# Autodesk Inventor assembly: Assembly6
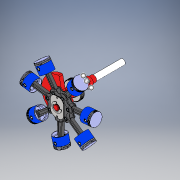
[picture p0: Inventor's stored thumbnail of the model, 180x180]
Saved by Autodesk Inventor 2018 (Build 220112000, 112)
## iProperties
Created: 2023-04-24
Part Number: Assembly6
Document SubType Name: Assembly
Designer: Habib Mohamed
Author: Habib Mohamed
## Documents named in this file (12)
- D:\Inventor\My projects\Rotary Engine\Assembly\Assembly6.iam
- D:\Inventor\My projects\Rotary Engine\Assembly\Assembly4 (Piston Sub Assembly).iam
- D:\Inventor\My projects\Rotary Engine\Component 2 (Connecting Rod Hub).ipt
- D:\Inventor\My projects\Rotary Engine\Component 31(Rod Axle).ipt
- D:\Inventor\My projects\Rotary Engine\Assembly\Assembly4 (Piston Sub Assembly Shrunk).iam
- D:\Inventor\My projects\Rotary Engine\Shaft.ipt
- D:\Inventor\My projects\Rotary Engine\Component 16 (Sun Wheel).ipt
- D:\Inventor\My projects\Rotary Engine\Component 17 (Feather Key).ipt
- D:\Inventor\My projects\Rotary Engine\Component 7 (Cover Plate).ipt
- C:\Users\Habib Mohamed\Documents\Inventor\Content Center Files\R2018\en-US\DIN 617 SKF(2)\DIN 617 SKF - SKF NA 4900 RS.ipt
- C:\Users\Habib Mohamed\Documents\Inventor\Content Center Files\R2018\en-US\DIN 6799\DIN 6799 - 9 10.ipt
- C:\Users\Habib Mohamed\Documents\Inventor\Content Center Files\R2018\en-US\DIN 6799\DIN 6799 - 10 11.ipt
## Components (21 placed, 11 different names)
1. Assembly4 (Piston Sub Assembly):1 [sub-assembly] — Mate:5, Mate:12
2. Component 2 (Connecting Rod Hub):1 — Mate:1, Mate:2, Mate:3, Mate:4, Mate:5, Mate:6, Mate:7, Mate:8, Mate:9, Mate:10, Mate:11, Mate:12, Mate:13, Mate:14, Mate:15, Mate:16, Mate:17, Mate:18, Mate:19, Mate:20, Flush:1, Flush:2, Flush:3, Flush:4, Flush:5, Mate:21, Mate:22, Mate:29, Mate:30, Flush:6, Mate:33, Mate:34
3. Component 31(Rod Axle):1 — Mate:18, Flush:1
4. Assembly4 (Piston Sub Assembly):2 [sub-assembly] — Mate:6, Mate:10
5. Assembly4 (Piston Sub Assembly):3 [sub-assembly] — Mate:7, Mate:11
6. Assembly4 (Piston Sub Assembly):4 [sub-assembly] — Mate:8, Mate:9
7. Assembly4 (Piston Sub Assembly):5 [sub-assembly] — Mate:4, Mate:13
8. Assembly4 (Piston Sub Assembly):6 [sub-assembly] — Mate:3, Mate:14
9. Assembly4 (Piston Sub Assembly Shrunk):1 [sub-assembly] — Mate:21, Mate:22
10. Component 31(Rod Axle):2 — Mate:16, Flush:3
11. Component 31(Rod Axle):3 — Mate:15, Flush:2
12. Component 31(Rod Axle):4 — Mate:20, Flush:5
13. Component 31(Rod Axle):5 — Mate:19, Flush:4
14. Component 31(Rod Axle):6 — Mate:17
15. Shaft:1 — Mate:23, Mate:24, Mate:25, Mate:26, Mate:27, Mate:28, Mate:29, Mate:31, Mate:32, Mate:35, Mate:37, Mate:38
16. Component 16 (Sun Wheel):1 — Mate:26, Mate:27, Mate:28
17. Component 17 (Feather Key):1 — Mate:23, Mate:24, Mate:25
18. Component 7 (Cover Plate):1 — Mate:32, Mate:33, Mate:34, Mate:36
19. DIN 617 SKF- with Inner Ring - NA 49...RS SKF NA 4900 RS:1 — Mate:30, Mate:31, Flush:6
20. DIN 6799 9:1 — Mate:35, Mate:36
21. DIN 6799 10:1 — Mate:37, Mate:38
## Relationships (44: Mate 38, Flush 6)
- Mate:1: Component 2 (Connecting Rod Hub):1
- Mate:2: Component 2 (Connecting Rod Hub):1
- Mate:3: Component 2 (Connecting Rod Hub):1 ↔ Assembly4 (Piston Sub Assembly):6
- Mate:4: Component 2 (Connecting Rod Hub):1 ↔ Assembly4 (Piston Sub Assembly):5
- Mate:5: Assembly4 (Piston Sub Assembly):1 ↔ Component 2 (Connecting Rod Hub):1
- Mate:6: Component 2 (Connecting Rod Hub):1 ↔ Assembly4 (Piston Sub Assembly):2
- Mate:7: Component 2 (Connecting Rod Hub):1 ↔ Assembly4 (Piston Sub Assembly):3
- Mate:8: Component 2 (Connecting Rod Hub):1 ↔ Assembly4 (Piston Sub Assembly):4
- Mate:9: Component 2 (Connecting Rod Hub):1 ↔ Assembly4 (Piston Sub Assembly):4
- Mate:10: Component 2 (Connecting Rod Hub):1 ↔ Assembly4 (Piston Sub Assembly):2
- Mate:11: Component 2 (Connecting Rod Hub):1 ↔ Assembly4 (Piston Sub Assembly):3
- Mate:12: Assembly4 (Piston Sub Assembly):1 ↔ Component 2 (Connecting Rod Hub):1
- Mate:13: Component 2 (Connecting Rod Hub):1 ↔ Assembly4 (Piston Sub Assembly):5
- Mate:14: Component 2 (Connecting Rod Hub):1 ↔ Assembly4 (Piston Sub Assembly):6
- Mate:15: Component 2 (Connecting Rod Hub):1 ↔ Component 31(Rod Axle):3
- Mate:16: Component 2 (Connecting Rod Hub):1 ↔ Component 31(Rod Axle):2
- Mate:17: Component 2 (Connecting Rod Hub):1 ↔ Component 31(Rod Axle):6
- Mate:18: Component 2 (Connecting Rod Hub):1 ↔ Component 31(Rod Axle):1
- Mate:19: Component 2 (Connecting Rod Hub):1 ↔ Component 31(Rod Axle):5
- Mate:20: Component 2 (Connecting Rod Hub):1 ↔ Component 31(Rod Axle):4
- Flush:1: Component 2 (Connecting Rod Hub):1 ↔ Component 31(Rod Axle):1
- Flush:2: Component 2 (Connecting Rod Hub):1 ↔ Component 31(Rod Axle):3
- Flush:3: Component 2 (Connecting Rod Hub):1 ↔ Component 31(Rod Axle):2
- Flush:4: Component 2 (Connecting Rod Hub):1 ↔ Component 31(Rod Axle):5
- Flush:5: Component 2 (Connecting Rod Hub):1 ↔ Component 31(Rod Axle):4
- Mate:21: Component 2 (Connecting Rod Hub):1 ↔ Assembly4 (Piston Sub Assembly Shrunk):1
- Mate:22: Component 2 (Connecting Rod Hub):1 ↔ Assembly4 (Piston Sub Assembly Shrunk):1
- Mate:23: Shaft:1 ↔ Component 17 (Feather Key):1
- Mate:24: Shaft:1 ↔ Component 17 (Feather Key):1
- Mate:25: Shaft:1 ↔ Component 17 (Feather Key):1
- Mate:26: Shaft:1 ↔ Component 16 (Sun Wheel):1
- Mate:27: Shaft:1 ↔ Component 16 (Sun Wheel):1
- Mate:28: Shaft:1 ↔ Component 16 (Sun Wheel):1
- Mate:29: Component 2 (Connecting Rod Hub):1 ↔ Shaft:1
- Mate:30: Component 2 (Connecting Rod Hub):1 ↔ DIN 617 SKF- with Inner Ring - NA 49...RS SKF NA 4900 RS:1
- Mate:31: Shaft:1 ↔ DIN 617 SKF- with Inner Ring - NA 49...RS SKF NA 4900 RS:1
- Flush:6: Component 2 (Connecting Rod Hub):1 ↔ DIN 617 SKF- with Inner Ring - NA 49...RS SKF NA 4900 RS:1
- Mate:32: Shaft:1 ↔ Component 7 (Cover Plate):1
- Mate:33: Component 2 (Connecting Rod Hub):1 ↔ Component 7 (Cover Plate):1
- Mate:34: Component 2 (Connecting Rod Hub):1 ↔ Component 7 (Cover Plate):1
- Mate:35: Shaft:1 ↔ DIN 6799 9:1
- Mate:36: Component 7 (Cover Plate):1 ↔ DIN 6799 9:1
- Mate:37: Shaft:1 ↔ DIN 6799 10:1
- Mate:38: Shaft:1 ↔ DIN 6799 10:1
